# Autodesk Inventor assembly: piping runs
(part 2 of 2)
PipeKey: v3#68e0b215-36a5-45d5-8e02-82e8f566f1ef#5
_ComponentInfo: <CS><C N="Pipe" R="2.120000" OR="2.120000" IR="1.800000" PL="PL" PartType="pipe" SymKey="" PN=""><CO N="1"><FE V="0"/><FD V="0"/><ET V="Threaded"/><NS V="1 1/4"/><MA V="1.500000"/><MI V="0.750000"/><WP X="0.000000" Y="0.000000" Z="10.000000"/><WA X="0.000000" Y="0.000000" Z="1.000000"/></CO><CO N="2"><FE V="0"/><FD V="1"/><ET V="Threaded"/><NS V="1 1/4"/><MA V="1.500000"/><MI V="0.750000"/><WP X="0.000000" Y="0.000000" Z="0.000000"/><WA X="0.000000" Y="0.000000" Z="1.000000"/></CO></C> <C N="Coupling" CW="5.000000" PartType="fitting" SymKey=""><CO N="1"><FE V="1"/><FD V="1"/><ET V="Threaded"/><NS V="1 1/4"/><MA V="1.500000"/><MI V="0.750000"/><WP X="5.000000" Y="0.000000" Z="0.000000"/><WA X="-1.000000" Y="0.000000" Z="0.000000"/></CO><CO N="2"><FE V="1"/><FD V="0"/><ET V="Threaded"/><NS V="1 1/4"/><MA V="1.500000"/><MI V="0.750000"/><WP X="-0.000000" Y="0.000000" Z="0.000000"/><WA X="-1.000000" Y="0.000000" Z="0.000000"/></CO></C> <C N="Elbow90" ER="3.000000" S1="4.500000" S2="4.500000" D1="1.500000" D2="1.500000" PartType="fitting" SymKey=""><CO N="1"><FE V="1"/><FD V="1"/><ET V="Threaded"/><NS V="1 1/4"/><MA V="1.500000"/><MI V="0.750000"/><WP X="4.500000" Y="0.000000" Z="2.600000"/><WA X="-1.000000" Y="0.000000" Z="-0.000000"/></CO><CO N="2"><FE V="1"/><FD V="0"/><ET V="Threaded"/><NS V="1 1/4"/><MA V="1.500000"/><MI V="0.750000"/><WP X="0.000000" Y="0.000000" Z="-1.900000"/><WA X="0.000000" Y="0.000000" Z="-1.000000"/></CO></C> <C N="Elbow45" ER="7.242641" S1="4.500000" S2="4.500000" D1="1.500000" D2="1.500000" PartType="fitting" SymKey=""><CO N="1"><FE V="1"/><FD V="1"/><ET V="Threaded"/><NS V="1 1/4"/><MA V="1.500000"/><MI V="0.750000"/><WP X="3.181981" Y="0.000000" Z="4.258936"/><WA X="-0.707107" Y="0.000000" Z="-0.707107"/></CO><CO N="2"><FE V="1"/><FD V="0"/><ET V="Threaded"/><NS V="1 1/4"/><MA V="1.500000"/><MI V="0.750000"/><WP X="-0.000000" Y="0.000000" Z="-3.423045"/><WA X="-0.000000" Y="0.000000" Z="-1.000000"/></CO></C> </CS>
FlangeKey: v3#24991861-26e3-4c21-a713-f46e314eddd5#10
Name: ASTM A 53/A 53M - Tuyau en acier à collet/soudé bout à bout
UseFlangsForCouplings: False
_ComponentInfo: <CS><C N="Pipe" R="8.413750" OR="8.413750" IR="7.702550" PL="PL" PartType="pipe" SymKey="" PN="ASTM A 53/A 53M Pipe 6 - Schedule 40"><CO N="1"><FE V="2"/><FD V="0"/><ET V="Welded"/><NS V="6"/><MA V="0.000000"/><MI V="0.000000"/><WP X="25.400000" Y="0.000000" Z="0.000000"/><WA X="1.000000" Y="0.000000" Z="0.000000"/></CO><CO N="2"><FE V="2"/><FD V="1"/><ET V="Welded"/><NS V="6"/><MA V="0.000000"/><MI V="0.000000"/><WP X="0.000000" Y="0.000000" Z="0.000000"/><WA X="1.000000" Y="0.000000" Z="0.000000"/></CO></C> <C N="Elbow90" ER="21.590000" S1="21.590000" S2="21.590000" D1="0.000000" D2="0.000000" PartType="fitting" SymKey="ELFL"><CO N="1"><FE V="2"/><FD V="1"/><ET V="Flanged"/><NS V="6"/><MA V="0.000000"/><MI V="0.000000"/><WP X="21.590000" Y="0.000000" Z="21.590000"/><WA X="-1.000000" Y="0.000000" Z="0.000000"/></CO><CO N="2"><FE V="2"/><FD V="0"/><ET V="Flanged"/><NS V="6"/><MA V="0.000000"/><MI V="0.000000"/><WP X="-0.000000" Y="0.000000" Z="-0.000000"/><WA X="-0.000000" Y="0.000000" Z="-1.000000"/></CO></C> <C N="Flange" CW="9.702800" PartType="fitting" SymKey="FLWN"><CO N="1"><FE V="2"/><FD V="1"/><ET V="Flanged"/><NS V="6"/><MA V="0.000000"/><MI V="0.000000"/><WP X="0.000000" Y="0.000000" Z="0.000000"/><WA X="1.000000" Y="0.000000" Z="0.000000"/></CO><CO N="2"><FE V="2"/><FD V="0"/><ET V="Butt Welded"/><NS V="6"/><MA V="0.000000"/><MI V="0.000000"/><WP X="9.702800" Y="0.000000" Z="0.000000"/><WA X="1.000000" Y="0.000000" Z="0.000000"/></CO></C> <C N="Gasket" CW="0.127000" PartType="fitting" SymKey=""><CO N="1"><FE V="2"/><FD V="1"/><ET V="Flanged"/><NS V="6"/><MA V="0.000000"/><MI V="0.000000"/><WP X="-0.000000" Y="0.127000" Z="0.000000"/><WA X="0.000000" Y="-1.000000" Z="0.000000"/></CO><CO N="2"><FE V="2"/><FD V="0"/><ET V="Flanged"/><NS V="6"/><MA V="0.000000"/><MI V="0.000000"/><WP X="-0.000000" Y="-0.000000" Z="0.000000"/><WA X="0.000000" Y="-1.000000" Z="0.000000"/></CO></C> </CS>
CouplingKey: v3#2b0a5189-15ae-469a-9b17-b414f6c6114b#7
Diameter: 2
Elbow45Key: v3#9d33c53f-93b2-4cb9-b7ec-24e123ef00cf#7
Elbow90Key: v3#2d4a59cf-155e-432e-9a7c-36306ddbf5a3#7
Name: Tuyau-GF / GF-Rohr - Tuyau avec raccords GF / Rohr und GF Fittings 2"
PipeKey: v3#68e0b215-36a5-45d5-8e02-82e8f566f1ef#7
_ComponentInfo: <CS><C N="Pipe" R="3.010000" OR="3.010000" IR="2.650000" PL="PL" PartType="pipe" SymKey="" PN=""><CO N="1"><FE V="0"/><FD V="0"/><ET V="Threaded"/><NS V="2"/><MA V="1.820000"/><MI V="0.910000"/><WP X="0.000000" Y="0.000000" Z="10.000000"/><WA X="0.000000" Y="0.000000" Z="1.000000"/></CO><CO N="2"><FE V="0"/><FD V="1"/><ET V="Threaded"/><NS V="2"/><MA V="1.820000"/><MI V="0.910000"/><WP X="0.000000" Y="0.000000" Z="0.000000"/><WA X="0.000000" Y="0.000000" Z="1.000000"/></CO></C> <C N="Coupling" CW="6.500000" PartType="fitting" SymKey=""><CO N="1"><FE V="1"/><FD V="1"/><ET V="Threaded"/><NS V="2"/><MA V="1.820000"/><MI V="0.910000"/><WP X="6.500000" Y="0.000000" Z="0.000000"/><WA X="-1.000000" Y="0.000000" Z="0.000000"/></CO><CO N="2"><FE V="1"/><FD V="0"/><ET V="Threaded"/><NS V="2"/><MA V="1.820000"/><MI V="0.910000"/><WP X="-0.000000" Y="0.000000" Z="0.000000"/><WA X="-1.000000" Y="0.000000" Z="0.000000"/></CO></C> <C N="Elbow90" ER="3.980000" S1="5.800000" S2="5.800000" D1="1.820000" D2="1.820000" PartType="fitting" SymKey=""><CO N="1"><FE V="1"/><FD V="1"/><ET V="Threaded"/><NS V="2"/><MA V="1.820000"/><MI V="0.910000"/><WP X="5.800000" Y="0.000000" Z="3.550000"/><WA X="-1.000000" Y="0.000000" Z="-0.000000"/></CO><CO N="2"><FE V="1"/><FD V="0"/><ET V="Threaded"/><NS V="2"/><MA V="1.820000"/><MI V="0.910000"/><WP X="-0.000000" Y="0.000000" Z="-2.250000"/><WA X="0.000000" Y="0.000000" Z="-1.000000"/></CO></C> <C N="Elbow45" ER="9.608570" S1="5.800000" S2="5.800000" D1="1.820000" D2="1.820000" PartType="fitting" SymKey=""><CO N="1"><FE V="1"/><FD V="1"/><ET V="Threaded"/><NS V="2"/><MA V="1.820000"/><MI V="0.910000"/><WP X="4.101219" Y="0.000000" Z="5.571677"/><WA X="-0.707107" Y="0.000000" Z="-0.707107"/></CO><CO N="2"><FE V="1"/><FD V="0"/><ET V="Threaded"/><NS V="2"/><MA V="1.820000"/><MI V="0.910000"/><WP X="-0.000000" Y="0.000000" Z="-4.329542"/><WA X="-0.000000" Y="0.000000" Z="-1.000000"/></CO></C> </CS>
EndFittingKey: v3#933069c9-73b6-4141-af99-628d4a97b2c2#1
Name: Tuyau flexible hydraulique - Connexion à brides SAE
StartFittingKey: v3#933069c9-73b6-4141-af99-628d4a97b2c2#1
_ComponentInfo: <CS><C N="Pipe" R="1.117600" OR="1.117600" IR="0.635000" PL="PL" PartType="" SymKey="" PN="Parker Hydraulic Hose - No Skive 1/2"><CO N="1"><FE V="0"/><FD V="0"/><ET V="Hose - Permanent"/><NS V="1/2"/><MA V="2.540000"/><MI V="0.508000"/><WP X="12.700000" Y="0.000000" Z="0.000000"/><WA X="1.000000" Y="0.000000" Z="0.000000"/></CO><CO N="2"><FE V="0"/><FD V="1"/><ET V="Hose - Permanent"/><NS V="1/2"/><MA V="2.540000"/><MI V="0.508000"/><WP X="0.000000" Y="0.000000" Z="0.000000"/><WA X="1.000000" Y="0.000000" Z="0.000000"/></CO></C><C N="StartFitting" PartType="MISC-HYGENIC" SymKey="ADMF"><CO N="1"><FE V="0"/><FD V="1"/><ET V="Flanged"/><NS V="1/2"/><MA V="0.000000"/><MI V="0.000000"/><WP X="0.000000" Y="0.000000" Z="0.000000"/><WA X="1.000000" Y="0.000000" Z="0.000000"/></CO><CO N="2"><FE V="1"/><FD V="0"/><ET V="Hose - Permanent"/><NS V="1/2"/><MA V="3.200000"/><MI V="3.200000"/><WP X="8.800000" Y="0.000000" Z="0.000000"/><WA X="1.000000" Y="0.000000" Z="0.000000"/></CO></C><C N="EndFitting" PartType="MISC-HYGENIC" SymKey="ADMF"><CO N="1"><FE V="0"/><FD V="1"/><ET V="Flanged"/><NS V="1/2"/><MA V="0.000000"/><MI V="0.000000"/><WP X="0.000000" Y="0.000000" Z="0.000000"/><WA X="1.000000" Y="0.000000" Z="0.000000"/></CO><CO N="2"><FE V="1"/><FD V="0"/><ET V="Hose - Permanent"/><NS V="1/2"/><MA V="3.200000"/><MI V="3.200000"/><WP X="8.800000" Y="0.000000" Z="0.000000"/><WA X="1.000000" Y="0.000000" Z="0.000000"/></CO></C></CS>
CouplingKey: v3#2b0a5189-15ae-469a-9b17-b414f6c6114b#6
Diameter: 1 1/2
Elbow45Key: v3#9d33c53f-93b2-4cb9-b7ec-24e123ef00cf#6
Elbow90Key: v3#2d4a59cf-155e-432e-9a7c-36306ddbf5a3#6
Name: Tuyau-GF / GF-Rohr - Tuyau avec raccords GF / Rohr und GF Fittings 1 1/2"
PipeKey: v3#68e0b215-36a5-45d5-8e02-82e8f566f1ef#6
_ComponentInfo: <CS><C N="Pipe" R="2.420000" OR="2.420000" IR="2.090000" PL="PL" PartType="pipe" SymKey="" PN=""><CO N="1"><FE V="0"/><FD V="0"/><ET V="Threaded"/><NS V="1 1/2"/><MA V="1.500000"/><MI V="0.750000"/><WP X="0.000000" Y="0.000000" Z="10.000000"/><WA X="0.000000" Y="0.000000" Z="1.000000"/></CO><CO N="2"><FE V="0"/><FD V="1"/><ET V="Threaded"/><NS V="1 1/2"/><MA V="1.500000"/><MI V="0.750000"/><WP X="0.000000" Y="0.000000" Z="0.000000"/><WA X="0.000000" Y="0.000000" Z="1.000000"/></CO></C> <C N="Coupling" CW="5.500000" PartType="fitting" SymKey=""><CO N="1"><FE V="1"/><FD V="1"/><ET V="Threaded"/><NS V="1 1/2"/><MA V="1.500000"/><MI V="0.750000"/><WP X="5.500000" Y="0.000000" Z="0.000000"/><WA X="-1.000000" Y="0.000000" Z="0.000000"/></CO><CO N="2"><FE V="1"/><FD V="0"/><ET V="Threaded"/><NS V="1 1/2"/><MA V="1.500000"/><MI V="0.750000"/><WP X="-0.000000" Y="0.000000" Z="0.000000"/><WA X="-1.000000" Y="0.000000" Z="0.000000"/></CO></C> <C N="Elbow90" ER="3.500000" S1="5.000000" S2="5.000000" D1="1.500000" D2="1.500000" PartType="fitting" SymKey=""><CO N="1"><FE V="1"/><FD V="1"/><ET V="Threaded"/><NS V="1 1/2"/><MA V="1.500000"/><MI V="0.750000"/><WP X="5.000000" Y="0.000000" Z="2.900000"/><WA X="-1.000000" Y="0.000000" Z="0.000000"/></CO><CO N="2"><FE V="1"/><FD V="0"/><ET V="Threaded"/><NS V="1 1/2"/><MA V="1.500000"/><MI V="0.750000"/><WP X="0.000000" Y="0.000000" Z="-2.100000"/><WA X="0.000000" Y="0.000000" Z="-1.000000"/></CO></C> <C N="Elbow45" ER="8.449747" S1="5.000000" S2="5.000000" D1="1.500000" D2="1.500000" PartType="fitting" SymKey=""><CO N="1"><FE V="1"/><FD V="1"/><ET V="Threaded"/><NS V="1 1/2"/><MA V="1.500000"/><MI V="0.750000"/><WP X="3.535534" Y="0.000000" Z="4.736753"/><WA X="-0.707107" Y="0.000000" Z="-0.707107"/></CO><CO N="2"><FE V="1"/><FD V="0"/><ET V="Threaded"/><NS V="1 1/2"/><MA V="1.500000"/><MI V="0.750000"/><WP X="-0.000000" Y="0.000000" Z="-3.798781"/><WA X="0.000000" Y="0.000000" Z="-1.000000"/></CO></C> </CS>
CouplingKey: v3#29993622-4c6a-437e-8b8c-43a0846f8735#1
Elbow45Key: v3#d7b5d569-4a12-4d65-ba55-12203d6ac7ed#1
Elbow90Key: v3#25d2a8db-6517-4627-a5a4-9d27e4d26b9b#1
Name: ASTM D 1785-ASTM D 2466 - Tuyau et fixations articulés en PVC
PipeKey: v3#4bf12049-4375-491b-8f13-d4ee0c517c57#1
_ComponentInfo: <CS><C N="Pipe" R="1.066800" IR="0.789940" PL="PL" PN="ASTM D 1785 Pipe 1/2 - Schedule 40"><CO N="1"><FE V="0"/><FD V="0"/><ET V="Jointed"/><NS V="1/2"/><MA V="2.540000"/><MI V="0.508000"/><WP X="127.000000" Y="0.000000" Z="0.000000"/><WA X="1.000000" Y="0.000000" Z="0.000000"/></CO><CO N="2"><FE V="0"/><FD V="1"/><ET V="Jointed"/><NS V="1/2"/><MA V="2.540000"/><MI V="0.508000"/><WP X="0.000000" Y="0.000000" Z="0.000000"/><WA X="1.000000" Y="0.000000" Z="0.000000"/></CO></C><C N="Coupling" CW="3.733165"><CO N="1"><FE V="1"/><FD V="0"/><ET V="Jointed"/><NS V="1/2"/><MA V="1.747520"/><MI V="0.349504"/><WP X="3.733165" Y="0.000000" Z="0.000000"/><WA X="1.000000" Y="0.000000" Z="0.000000"/></CO><CO N="2"><FE V="1"/><FD V="1"/><ET V="Jointed"/><NS V="1/2"/><MA V="1.747520"/><MI V="0.349504"/><WP X="0.000000" Y="0.000000" Z="0.000000"/><WA X="1.000000" Y="0.000000" Z="0.000000"/></CO></C><C N="Elbow90" ER="1.270000" S1="3.017520" S2="3.017520" D1="1.747520" D2="1.747520"><CO N="1"><FE V="1"/><FD V="1"/><ET V="Jointed"/><NS V="1/2"/><MA V="1.747520"/><MI V="0.349504"/><WP X="3.017520" Y="0.000000" Z="3.017520"/><WA X="-1.000000" Y="0.000000" Z="-0.000000"/></CO><CO N="2"><FE V="1"/><FD V="1"/><ET V="Jointed"/><NS V="1/2"/><MA V="1.747520"/><MI V="0.349504"/><WP X="0.000000" Y="0.000000" Z="0.000000"/><WA X="0.000000" Y="0.000000" Z="1.000000"/></CO></C><C N="Elbow45" ER="1.533026" S1="2.382520" S2="2.382520" D1="1.747520" D2="1.747520"><CO N="1"><FE V="1"/><FD V="1"/><ET V="Jointed"/><NS V="1/2"/><MA V="1.747520"/><MI V="0.349504"/><WP X="1.684696" Y="0.000000" Z="4.067216"/><WA X="-0.707107" Y="0.000000" Z="-0.707107"/></CO><CO N="2"><FE V="1"/><FD V="1"/><ET V="Jointed"/><NS V="1/2"/><MA V="1.747520"/><MI V="0.349504"/><WP X="0.000000" Y="0.000000" Z="0.000000"/><WA X="0.000000" Y="0.000000" Z="1.000000"/></CO></C></CS>
count: 66
Refkey_Axis1_Context: 2|0|0|0|1|0|0|0|
Refkey_Axis1: 6|0|0|0|44|0|0|0|78|0|65|0|77|0|69|0|83|0|10|0|67|0|111|0|108|0|111|0|114|0|115|0|10|0|49|0|58|0|10|0|10|0|69|0|78|0|68|0|10|0|0|0|
Refkey_Axis2_Context: 2|0|0|0|1|0|0|0|
Refkey_Axis2: 6|0|0|0|88|0|0|0|78|0|65|0|77|0|69|0|83|0|10|0|67|0|111|0|108|0|111|0|114|0|115|0|10|0|49|0|58|0|82|0|111|0|117|0|116|0|101|0|32|0|85|0|73|0|32|0|84|0|111|0|111|0|108|0|32|0|40|0|65|0|120|0|105|0|115|0|32|0|50|0|41|0|10|0|10|0|69|0|78|0|68|0|10|0|0|0|
Refkey_Axis3_Context: 2|0|0|0|1|0|0|0|
Refkey_Axis3: 6|0|0|0|88|0|0|0|78|0|65|0|77|0|69|0|83|0|10|0|67|0|111|0|108|0|111|0|114|0|115|0|10|0|49|0|58|0|82|0|111|0|117|0|116|0|101|0|32|0|85|0|73|0|32|0|84|0|111|0|111|0|108|0|32|0|40|0|65|0|120|0|105|0|115|0|32|0|51|0|41|0|10|0|10|0|69|0|78|0|68|0|10|0|0|0|
Refkey_Ext_Context: 2|0|0|0|1|0|0|0|
Refkey_Ext: 6|0|0|0|92|0|0|0|78|0|65|0|77|0|69|0|83|0|10|0|67|0|111|0|108|0|111|0|114|0|115|0|10|0|49|0|58|0|82|0|111|0|117|0|116|0|101|0|32|0|85|0|73|0|32|0|84|0|111|0|111|0|108|0|32|0|40|0|69|0|120|0|116|0|101|0|110|0|100|0|101|0|114|0|41|0|10|0|10|0|69|0|78|0|68|0|10|0|0|0|
Refkey_Snap_Context: 2|0|0|0|1|0|0|0|
Refkey_Snap: 6|0|0|0|84|0|0|0|78|0|65|0|77|0|69|0|83|0|10|0|67|0|111|0|108|0|111|0|114|0|115|0|10|0|49|0|58|0|82|0|111|0|117|0|116|0|101|0|32|0|85|0|73|0|32|0|84|0|111|0|111|0|108|0|32|0|40|0|83|0|110|0|97|0|112|0|41|0|10|0|10|0|69|0|78|0|68|0|10|0|0|0|
CouplingKey: v3#d2599e7a-1865-48da-a234-5418a1cd5dfe#3
Elbow45Key: v3#6ce5b1be-37aa-4928-b23a-0df64e6ddf38#2
Elbow90Key: v3#9fba244e-81ed-4fc6-a9ac-7eb372fa3ffe#3
Name: DIN 2458/DIN EN 10242 - Tuyau en acier fileté et fixations en fer
PipeKey: v3#d689fd5f-ac5a-46d7-a883-3089b2f6e0a4#28
Schedule: ID=12.3
_ComponentInfo: <CS><C N="Pipe" R="1.065000" IR="0.615000" PL="PL" PN="DIN 2458 Pipe with Threaded Ends 21.3 x 4.5"><CO N="1"><FE V="0"/><FD V="1"/><ET V="Threaded"/><NS V="1/2"/><MA V="1.372000"/><MI V="0.274400"/><WP X="25.000000" Y="0.000000" Z="-0.000000"/><WA X="-1.000000" Y="0.000000" Z="0.000000"/></CO><CO N="2"><FE V="0"/><FD V="0"/><ET V="Threaded"/><NS V="1/2"/><MA V="1.372000"/><MI V="0.274400"/><WP X="-0.000000" Y="0.000000" Z="-0.000000"/><WA X="-1.000000" Y="0.000000" Z="0.000000"/></CO></C><C N="Coupling" CW="3.600000"><CO N="1"><FE V="1"/><FD V="1"/><ET V="Threaded"/><NS V="1/2"/><MA V="1.300000"/><MI V="0.260000"/><WP X="0.000000" Y="0.000000" Z="0.000000"/><WA X="1.000000" Y="0.000000" Z="0.000000"/></CO><CO N="2"><FE V="1"/><FD V="0"/><ET V="Threaded"/><NS V="1/2"/><MA V="1.300000"/><MI V="0.260000"/><WP X="3.600000" Y="0.000000" Z="0.000000"/><WA X="1.000000" Y="0.000000" Z="0.000000"/></CO></C><C N="Elbow90" ER="4.200000" S1="5.500000" S2="5.500000" D1="1.300000" D2="1.300000"><CO N="1"><FE V="1"/><FD V="0"/><ET V="Threaded"/><NS V="1/2"/><MA V="1.300000"/><MI V="0.260000"/><WP X="-0.000000" Y="0.000000" Z="-0.000000"/><WA X="-0.000000" Y="0.000000" Z="-1.000000"/></CO><CO N="2"><FE V="1"/><FD V="1"/><ET V="Threaded"/><NS V="1/2"/><MA V="1.300000"/><MI V="0.260000"/><WP X="5.500000" Y="0.000000" Z="5.500000"/><WA X="-1.000000" Y="0.000000" Z="0.000000"/></CO></C><C N="Elbow45" ER="5.552691" S1="3.600000" S2="3.600000" D1="1.300000" D2="1.300000"><CO N="1"><FE V="1"/><FD V="1"/><ET V="Threaded"/><NS V="1/2"/><MA V="1.300000"/><MI V="0.260000"/><WP X="2.545584" Y="0.000000" Z="6.145584"/><WA X="-0.707107" Y="0.000000" Z="-0.707107"/></CO><CO N="2"><FE V="1"/><FD V="0"/><ET V="Threaded"/><NS V="1/2"/><MA V="1.300000"/><MI V="0.260000"/><WP X="-0.000000" Y="0.000000" Z="-0.000000"/><WA X="-0.000000" Y="0.000000" Z="-1.000000"/></CO></C></CS>
CouplingKey: v3#2b0a5189-15ae-469a-9b17-b414f6c6114b#2
Elbow45Key: v3#9d33c53f-93b2-4cb9-b7ec-24e123ef00cf#2
Elbow90Key: v3#2d4a59cf-155e-432e-9a7c-36306ddbf5a3#2
Name: Tuyau-GF / GF-Rohr - Tuyau avec raccords GF / Rohr und GF Fittings 1/2"
PipeKey: v3#68e0b215-36a5-45d5-8e02-82e8f566f1ef#2
_ComponentInfo: <CS><C N="Pipe" R="1.070000" OR="1.070000" IR="0.805000" PL="PL" PartType="pipe" SymKey="" PN=""><CO N="1"><FE V="0"/><FD V="0"/><ET V="Threaded"/><NS V="1/2"/><MA V="1.000000"/><MI V="0.500000"/><WP X="0.000000" Y="0.000000" Z="10.000000"/><WA X="0.000000" Y="0.000000" Z="1.000000"/></CO><CO N="2"><FE V="0"/><FD V="1"/><ET V="Threaded"/><NS V="1/2"/><MA V="1.000000"/><MI V="0.500000"/><WP X="0.000000" Y="0.000000" Z="0.000000"/><WA X="0.000000" Y="0.000000" Z="1.000000"/></CO></C> <C N="Coupling" CW="3.600000" PartType="fitting" SymKey=""><CO N="1"><FE V="1"/><FD V="1"/><ET V="Threaded"/><NS V="1/2"/><MA V="1.000000"/><MI V="0.500000"/><WP X="3.600000" Y="0.000000" Z="0.000000"/><WA X="-1.000000" Y="0.000000" Z="0.000000"/></CO><CO N="2"><FE V="1"/><FD V="0"/><ET V="Threaded"/><NS V="1/2"/><MA V="1.000000"/><MI V="0.500000"/><WP X="-0.000000" Y="0.000000" Z="0.000000"/><WA X="-1.000000" Y="0.000000" Z="0.000000"/></CO></C> <C N="Elbow90" ER="1.800000" S1="2.800000" S2="2.800000" D1="1.000000" D2="1.000000" PartType="fitting" SymKey=""><CO N="1"><FE V="1"/><FD V="1"/><ET V="Threaded"/><NS V="1/2"/><MA V="1.000000"/><MI V="0.500000"/><WP X="2.800000" Y="0.000000" Z="1.500000"/><WA X="-1.000000" Y="0.000000" Z="0.000000"/></CO><CO N="2"><FE V="1"/><FD V="0"/><ET V="Threaded"/><NS V="1/2"/><MA V="1.000000"/><MI V="0.500000"/><WP X="-0.000000" Y="0.000000" Z="-1.300000"/><WA X="0.000000" Y="0.000000" Z="-1.000000"/></CO></C> <C N="Elbow45" ER="4.345584" S1="2.800000" S2="2.800000" D1="1.000000" D2="1.000000" PartType="fitting" SymKey=""><CO N="1"><FE V="1"/><FD V="1"/><ET V="Threaded"/><NS V="1/2"/><MA V="1.000000"/><MI V="0.500000"/><WP X="1.979899" Y="0.000000" Z="2.601219"/><WA X="-0.707107" Y="0.000000" Z="-0.707107"/></CO><CO N="2"><FE V="1"/><FD V="0"/><ET V="Threaded"/><NS V="1/2"/><MA V="1.000000"/><MI V="0.500000"/><WP X="-0.000000" Y="0.000000" Z="-2.178680"/><WA X="-0.000000" Y="0.000000" Z="-1.000000"/></CO></C> </CS>
Author: Autodesk
## Documents named in this file (1)
- C:\Users\Public\Documents\Autodesk\Inventor 2019\Design Data\Tube & Pipe\fr-FR\piping runs.iam
